# Autodesk Inventor assembly: controlunit
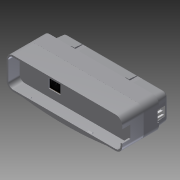
[picture p0: Inventor's stored thumbnail of the model, 180x180]
Saved by Autodesk Inventor 2014 (Build 180170000, 170)
## iProperties
Created: 2014-04-06
Part Number: controlunit
Document SubType Name: Assembly
Designer: Tyler
Author: Tyler
## Documents named in this file (4)
- C:\Users\Tyler\Documents\ft8900cad\controlunit.iam
- C:\Users\Tyler\Documents\ft8900cad\case_rear.ipt
- C:\Users\Tyler\Documents\ft8900cad\PCB\PCB.iam
- C:\Users\Tyler\Documents\ft8900cad\case_front.ipt
## Components (3 placed, 3 different names)
1. case_rear:1 — Mate:1, Mate:2, Mate:3, Flush:1, Flush:2, Mate:4
2. PCB:1 [sub-assembly] — Mate:1, Mate:2, Mate:3
3. case_front:1 — Flush:1, Flush:2, Mate:4
## Relationships (6: Mate 4, Flush 2)
- Mate:1: case_rear:1 ↔ PCB:1
- Mate:2: case_rear:1 ↔ PCB:1
- Mate:3: case_rear:1 ↔ PCB:1
- Flush:1: case_rear:1 ↔ case_front:1
- Flush:2: case_rear:1 ↔ case_front:1
- Mate:4: case_rear:1 ↔ case_front:1
